# Autodesk Inventor assembly: side_senzor
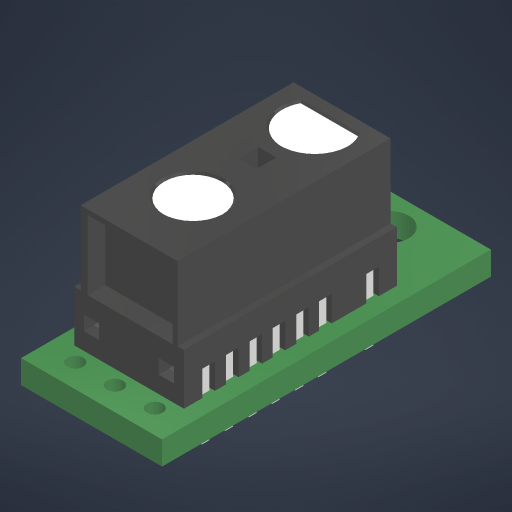
[picture p0: Inventor's stored thumbnail of the model, 512x512]
Saved by Autodesk Inventor 2024 (Build 280153000, 153)
## iProperties
Created: 2024-02-28
Part Number: side_senzor
Document SubType Name: Assembly
Designer: Simak
Author: Simak
## Documents named in this file (3)
- C:\Users\Simak\OneDrive\Dokumenty\GitHub\RoboCop\- 3D -\el._parts\SensorSharpDigital\side_senzor.iam
- C:\Users\Simak\OneDrive\Dokumenty\GitHub\RoboCop\- 3D -\el._parts\SensorSharpDigital\Base\Base.ipt
- C:\Users\Simak\OneDrive\Dokumenty\GitHub\RoboCop\- 3D -\el._parts\SensorSharpDigital\GP2Y0D810Z0F sharp\GP2Y0D810Z0F sharp.ipt
## Components (2 placed, 2 different names)
1. Base:1 — Proti sobě:1, Stejný směr:1, Stejný směr:2
2. GP2Y0D810Z0F sharp:1 — Proti sobě:1, Stejný směr:1, Stejný směr:2
## Relationships (3: Flush 2, Mate 1)
- Proti sobě:1 [Mate]: Base:1 ↔ GP2Y0D810Z0F sharp:1
- Stejný směr:1 [Flush] (2.4 mm): Base:1 ↔ GP2Y0D810Z0F sharp:1
- Stejný směr:2 [Flush] (1 mm): Base:1 ↔ GP2Y0D810Z0F sharp:1
